# Autodesk Inventor assembly: 775pro_3_1-2inHex
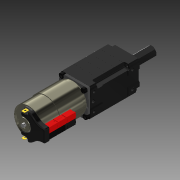
[picture p0: Inventor's stored thumbnail of the model, 180x180]
Saved by Autodesk Inventor 2022 (Build 260153000, 153)
## iProperties
Created: 2018-08-19
Part Number: 775pro_3_1-2inHex
Document SubType Name: Assembly
Mass: 1123.04 g
Surface Area: 1203.25 cm^2
Volume: 285.054 cm^3
Density: 3.93975 g/cm^3
## Documents named in this file (10)
- C:\Users\Cal\Desktop\Robotics\Design\Collaborative\Collaborative Parts Library\General Gearboxes\Planetaries\Versaplanetary\VersaPlanetary\775pro, 3 Stages, 1-2in Hex Output.iam
- C:\Users\Cal\Desktop\Robotics\Design\Collaborative\Collaborative Parts Library\General Gearboxes\Planetaries\Versaplanetary\Intermediate Stages\Ring Gear.ipt
- C:\Users\Cal\Desktop\Robotics\Design\Collaborative\Collaborative Parts Library\General Gearboxes\Planetaries\Versaplanetary\V2 Stages\V2 Input Stage.iam
- C:\Users\Cal\Desktop\Robotics\Design\Collaborative\Collaborative Parts Library\General Gearboxes\Planetaries\Versaplanetary\Screws\8-32 x 2.75in Screw.ipt
- C:\Users\Cal\Desktop\Robotics\Design\Collaborative\Collaborative Parts Library\Power Transfer\Bearings and Bushings\Bearings\6902ZZ.ipt
- E:\Middleton Robotics\Collaborative Robots\Colaborative Part Library\General Gearboxes\Planetaries\Versaplanetary\V2 Stages\V2 Output Stage.iam
- E:\Middleton Robotics\Collaborative Robots\Collaborative Part Library\Power Transfer\Bearings.ipt
- C:\Users\Cal\Desktop\Robotics\Design\Collaborative\Collaborative Parts Library\General Gearboxes\Planetaries\Versaplanetary\V2 Stages\V2 Output Stage\VP V2 Output Stage 1-2in Hex.iam
- C:\Users\Cal\Desktop\Robotics\Design\Collaborative\Collaborative Parts Library\General Gearboxes\Planetaries\Versaplanetary\V2 Stages\V2 Input Stage\VP 775pro Input.iam
- C:\Users\Cal\Desktop\Robotics\Design\Collaborative\Collaborative Parts Library\General Gearboxes\Planetaries\Versaplanetary\VersaPlanetary.iam
## Components (9 placed, 7 different names)
1. VP V2 Output Stage 1-2in Hex:1 [sub-assembly] — Insert:1, Flush:3, Flush:6, 3StageBasicInputMate2, Insert:25
2. Ring Gear 1 — Insert:1, Insert:2, Flush:1, Flush:3
3. Ring Gear 2 — Insert:2, Insert:3, Flush:1, Flush:2, Flush:6
4. Ring Gear 3 — Insert:3, Flush:2, 3StageBasicInputMate1
5. VP 775pro Input:1 [sub-assembly] — 3StageBasicInputMate1, 3StageBasicInputMate2, Insert:14, Insert:15
6. 8-32 x 2.75in Screw:1 — Insert:14
7. 8-32 x 2.75in Screw:2 — Insert:15
8. 6902ZZ:1
9. 6902ZZ:2 — Insert:25
## Relationships (12: Insert 7, Flush 5)
- Insert:1: VP V2 Output Stage 1-2in Hex:1 ↔ Ring Gear 1
- Insert:2: Ring Gear 1 ↔ Ring Gear 2
- Insert:3: Ring Gear 2 ↔ Ring Gear 3
- Flush:1: Ring Gear 1 ↔ Ring Gear 2
- Flush:2: Ring Gear 2 ↔ Ring Gear 3
- Flush:3: VP V2 Output Stage 1-2in Hex:1 ↔ Ring Gear 1
- Flush:6: VP V2 Output Stage 1-2in Hex:1 ↔ Ring Gear 2
- 3StageBasicInputMate1 [Insert]: Ring Gear 3 ↔ VP 775pro Input:1
- 3StageBasicInputMate2 [Flush]: VP V2 Output Stage 1-2in Hex:1 ↔ VP 775pro Input:1
- Insert:14: VP 775pro Input:1 ↔ 8-32 x 2.75in Screw:1
- Insert:15: VP 775pro Input:1 ↔ 8-32 x 2.75in Screw:2
- Insert:25: VP V2 Output Stage 1-2in Hex:1 ↔ 6902ZZ:2
